# Autodesk Inventor assembly: EstacaoAutomatizada
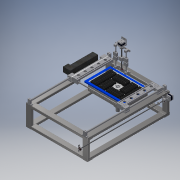
[picture p0: Inventor's stored thumbnail of the model, 180x180]
Saved by Autodesk Inventor 2018 (Build 220112000, 112)
## iProperties
Created: 2018-09-20
Part Number: EstacaoAutomatizada
Material: Genérico
Document SubType Name: Assembly
Designer: Georgines
_SolveAssemblyDoc: Frame Generator Solve Assembly
_Version: 15.0.0
Author: Georgines
## Documents named in this file (12)
- C:\Users\Usuario\Desktop\Estação BGA\Peças 3D\EstacaoAutomatizada.iam
- C:\Users\Usuario\Desktop\Estação BGA\Peças 3D\FrameBase.ipt
- C:\Users\Usuario\Desktop\Estação BGA\Peças 3D\EstacaoAutomatizada\Frame\Frame0001.iam
- C:\Users\Usuario\Desktop\Estação BGA\Peças 3D\Sk16.ipt
- C:\Users\Usuario\Desktop\Estação BGA\Peças 3D\GuiaLinear_16mmx800mm.ipt
- C:\Users\Usuario\Desktop\Estação BGA\Peças 3D\mesa_suporte_de_placa_automatica.iam
- C:\Users\Usuario\Desktop\Estação BGA\Peças 3D\SBR16UU.iam
- C:\Users\Usuario\Desktop\Estação BGA\Peças 3D\mesa_aquecimento_fresamento.iam
- C:\Users\Usuario\Desktop\Estação BGA\Peças 3D\cabeça_inferior.iam
- C:\Users\Usuario\Desktop\Estação BGA\Peças 3D\carro_linear.iam
- C:\Users\Usuario\Desktop\Estação BGA\Peças 3D\EixoY.iam
- C:\Users\Usuario\Desktop\Estação BGA\Peças 3D\ventilador_tangencial_referencia.ipt
## Components (18 placed, 11 different names)
1. FrameBase:1
2. Frame0001:1 [sub-assembly] — Coincidência:5, Coincidência:6, Alinhamento:18, Alinhamento:19, Coincidência:14, Alinhamento:20
3. Sk16:1 — Coincidência:1, Alinhamento:1, Alinhamento:3, Coincidência:6, Alinhamento:17, Alinhamento:18, Alinhamento:19
4. Sk16:2 — Alinhamento:2, Coincidência:2, Alinhamento:3, Coincidência:13
5. Sk16:3 — Coincidência:3, Alinhamento:4, Alinhamento:5, Coincidência:5, Alinhamento:17
6. Sk16:4 — Coincidência:4, Alinhamento:5, Alinhamento:6
7. GuiaLinear_16mmx800mm:1 — Coincidência:1, Alinhamento:1, Alinhamento:2, Coincidência:2, Coincidência:7, Coincidência:8
8. GuiaLinear_16mmx800mm:2 — Coincidência:3, Coincidência:4, Alinhamento:4, Alinhamento:6, Coincidência:9, Coincidência:10
9. mesa_suporte_de_placa_automatica:1 [sub-assembly] — Coincidência:11, Coincidência:12, Alinhamento:11, Alinhamento:12, Alinhamento:13, Alinhamento:14, Alinhamento:15, Alinhamento:16
10. SBR16UU:1 [sub-assembly] — Coincidência:7, Alinhamento:9, Coincidência:11, Alinhamento:13
11. SBR16UU:2 [sub-assembly] — Coincidência:8, Alinhamento:9, Alinhamento:12, Alinhamento:16, Coincidência:13
12. SBR16UU:3 [sub-assembly] — Coincidência:9, Alinhamento:10, Alinhamento:15
13. SBR16UU:4 [sub-assembly] — Coincidência:10, Alinhamento:10, Coincidência:12, Alinhamento:11, Alinhamento:14
14. mesa_aquecimento_fresamento:1 [sub-assembly]
15. cabeça_inferior:1 [sub-assembly]
16. carro_linear:1 [sub-assembly]
17. EixoY:1 [sub-assembly] — Coincidência:14, Alinhamento:20
18. ventilador_tangencial_referencia:1
## Relationships (32: Flush 18, Mate 14)
- Coincidência:1 [Mate]: Sk16:1 ↔ GuiaLinear_16mmx800mm:1
- Alinhamento:1 [Flush]: Sk16:1 ↔ GuiaLinear_16mmx800mm:1
- Alinhamento:2 [Flush]: Sk16:2 ↔ GuiaLinear_16mmx800mm:1
- Coincidência:2 [Mate]: Sk16:2 ↔ GuiaLinear_16mmx800mm:1
- Alinhamento:3 [Flush]: Sk16:1 ↔ Sk16:2
- Coincidência:3 [Mate]: Sk16:3 ↔ GuiaLinear_16mmx800mm:2
- Coincidência:4 [Mate]: Sk16:4 ↔ GuiaLinear_16mmx800mm:2
- Alinhamento:4 [Flush]: Sk16:3 ↔ GuiaLinear_16mmx800mm:2
- Alinhamento:5 [Flush]: Sk16:3 ↔ Sk16:4
- Alinhamento:6 [Flush]: Sk16:4 ↔ GuiaLinear_16mmx800mm:2
- Coincidência:5 [Mate]: Frame0001:1 ↔ Sk16:3
- Coincidência:6 [Mate]: Frame0001:1 ↔ Sk16:1
- Coincidência:7 [Mate]: GuiaLinear_16mmx800mm:1 ↔ SBR16UU:1
- Coincidência:8 [Mate]: GuiaLinear_16mmx800mm:1 ↔ SBR16UU:2
- Coincidência:9 [Mate]: GuiaLinear_16mmx800mm:2 ↔ SBR16UU:3
- Coincidência:10 [Mate]: GuiaLinear_16mmx800mm:2 ↔ SBR16UU:4
- Alinhamento:9 [Flush]: SBR16UU:1 ↔ SBR16UU:2
- Alinhamento:10 [Flush]: SBR16UU:3 ↔ SBR16UU:4
- Coincidência:11 [Mate]: mesa_suporte_de_placa_automatica:1 ↔ SBR16UU:1
- Coincidência:12 [Mate]: mesa_suporte_de_placa_automatica:1 ↔ SBR16UU:4
- Alinhamento:11 [Flush]: mesa_suporte_de_placa_automatica:1 ↔ SBR16UU:4
- Alinhamento:12 [Flush]: mesa_suporte_de_placa_automatica:1 ↔ SBR16UU:2
- Alinhamento:13 [Flush]: mesa_suporte_de_placa_automatica:1 ↔ SBR16UU:1
- Alinhamento:14 [Flush]: mesa_suporte_de_placa_automatica:1 ↔ SBR16UU:4
- Alinhamento:15 [Flush]: mesa_suporte_de_placa_automatica:1 ↔ SBR16UU:3
- Alinhamento:16 [Flush]: mesa_suporte_de_placa_automatica:1 ↔ SBR16UU:2
- Alinhamento:17 [Flush]: Sk16:1 ↔ Sk16:3
- Alinhamento:18 [Flush]: Frame0001:1 ↔ Sk16:1
- Alinhamento:19 [Flush] (5 mm): Frame0001:1 ↔ Sk16:1
- Coincidência:13 [Mate]: Sk16:2 ↔ SBR16UU:2
- Coincidência:14 [Mate]: Frame0001:1 ↔ EixoY:1
- Alinhamento:20 [Flush]: Frame0001:1 ↔ EixoY:1
